# Autodesk Inventor assembly: Frame_Gantry
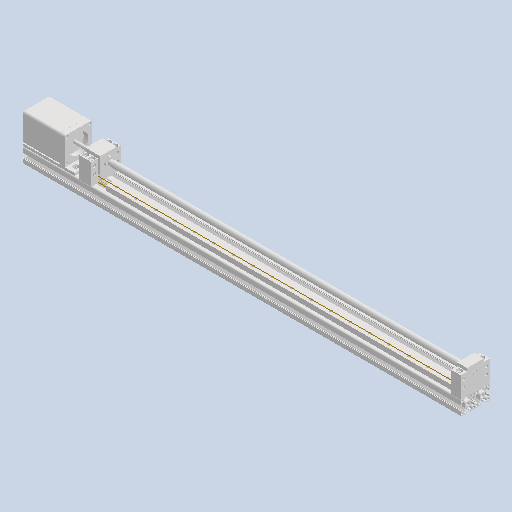
[picture p0: Inventor's stored thumbnail of the model, 512x512]
Saved by Autodesk Inventor 2023 (Build 270158000, 158)
## iProperties
Created: 2022-04-29
Part Number: Frame_Gantry
Document SubType Name: Assembly
Designer: plebbb
Author: plebbb
## Documents named in this file (10)
- D:\Users\plebbb\Desktop\CNC_Project\Frame_Gantry_Reverse.iam
- D:\Users\plebbb\Desktop\CNC_Project\MGN15H.iam
- D:\Users\plebbb\Desktop\CNC_Project\SFU1204.iam
- D:\Users\plebbb\Desktop\CNC_Project\BK10_Frame.ipt
- D:\Users\plebbb\Desktop\CNC_Project\BK10_3030_Mount.ipt
- D:\Users\plebbb\Desktop\CNC_Project\BF10.ipt
- D:\Users\plebbb\Desktop\CNC_Project\BF10_3030_Mount.ipt
- D:\Users\plebbb\Desktop\CNC_Project\Nema23.ipt
- D:\Users\plebbb\Desktop\CNC_Project\3030_Extrusion.ipt
- D:\Users\plebbb\Desktop\CNC_Project\NEMA23_Mount.ipt
## Components (10 placed, 9 different names)
1. MGN15H:1 [sub-assembly] — Mate:22, Flush:13, Mate:35
2. SFU1204:1 [sub-assembly] — Mate:6, Mate:7, Mate:27, Flush:10, Mate:32, Mate:33
3. BK10 — Mate:6, Mate:7, Mate:19, Mate:20, Angle:2, Flush:14
4. BK10_3030_Mount:1 — Mate:19, Mate:20, Mate:22, Mate:36
5. BF10:1 — Mate:24, Mate:25, Mate:27, Mate:28, Flush:10, Flush:15
6. BF10_3030_Mount:1 — Mate:24, Mate:25, Mate:28, Mate:37, Flush:16
7. Nema23:1 — Mate:32, Angle:2, Mate:33, Mate:39, Mate:40, Mate:41
8. 3030_Extrusion:1 — Mate:34, Flush:11, Flush:12, Mate:36, Mate:37, Flush:13
9. 3030_Extrusion:2 — Mate:34, Flush:11, Flush:12, Mate:35, Flush:14, Flush:15, Flush:16
10. NEMA23_Mount:1 — Mate:39, Mate:40, Mate:41
## Relationships (26: Mate 18, Flush 7, Angle 1)
- Mate:6: SFU1204:1 ↔ BK10
- Mate:7: SFU1204:1 ↔ BK10
- Mate:19: BK10 ↔ BK10_3030_Mount:1
- Mate:20: BK10 ↔ BK10_3030_Mount:1
- Mate:22 (22 mm): MGN15H:1 ↔ BK10_3030_Mount:1
- Mate:24: BF10:1 ↔ BF10_3030_Mount:1
- Mate:25: BF10:1 ↔ BF10_3030_Mount:1
- Mate:27: SFU1204:1 ↔ BF10:1
- Mate:28: BF10:1 ↔ BF10_3030_Mount:1
- Flush:10: SFU1204:1 ↔ BF10:1
- Mate:32: SFU1204:1 ↔ Nema23:1
- Angle:2 (0 deg): BK10 ↔ Nema23:1
- Mate:33: SFU1204:1 ↔ Nema23:1
- Mate:34: 3030_Extrusion:1 ↔ 3030_Extrusion:2
- Flush:11: 3030_Extrusion:1 ↔ 3030_Extrusion:2
- Flush:12: 3030_Extrusion:1 ↔ 3030_Extrusion:2
- Flush:13 (7.5 mm): MGN15H:1 ↔ 3030_Extrusion:1
- Mate:35: MGN15H:1 ↔ 3030_Extrusion:2
- Mate:36: BK10_3030_Mount:1 ↔ 3030_Extrusion:1
- Mate:37: BF10_3030_Mount:1 ↔ 3030_Extrusion:1
- Flush:14: BK10 ↔ 3030_Extrusion:2
- Flush:15: BF10:1 ↔ 3030_Extrusion:2
- Flush:16: BF10_3030_Mount:1 ↔ 3030_Extrusion:2
- Mate:39: Nema23:1 ↔ NEMA23_Mount:1
- Mate:40: Nema23:1 ↔ NEMA23_Mount:1
- Mate:41: Nema23:1 ↔ NEMA23_Mount:1
